# Autodesk Inventor assembly: Assembly2
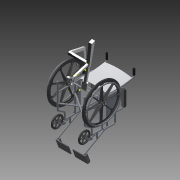
[picture p0: Inventor's stored thumbnail of the model, 180x180]
Saved by Autodesk Inventor 2017 (Build 210142000, 142)
## iProperties
Created: 2021-04-21
Part Number: Assembly2
Document SubType Name: Assembly
Designer: Anthony
Author: Anthony
## Documents named in this file (8)
- C:\Users\ANTHONY\Documents\Inventor\wheelchair project\Assembly2.iam
- C:\Users\ANTHONY\Documents\Inventor\wheelchair project\wheelchair.ipt
- C:\Users\ANTHONY\Documents\Inventor\wheelchair project\sweep.ipt
- C:\Users\ANTHONY\Documents\Inventor\wheelchair project\grip.ipt
- C:\Users\ANTHONY\Documents\Inventor\wheelchair project\wheel2.ipt
- C:\Users\ANTHONY\Documents\Inventor\wheelchair project\grip - Copy1.ipt
- C:\Users\ANTHONY\Documents\Inventor\wheelchair project\pin.ipt
- C:\Users\ANTHONY\Documents\Inventor\wheelchair project\handle.ipt
## Components (7 placed, 7 different names)
1. wheelchair:1
2. sweep:2
3. grip:1
4. wheel2:1
5. grip - Copy1:1 — Insert:1
6. pin:1 — Insert:1
7. handle:1
## Relationships (1: Insert 1)
- Insert:1 (-33 mm): grip - Copy1:1 ↔ pin:1
